# Autodesk Inventor assembly: Complete_leg_assembly
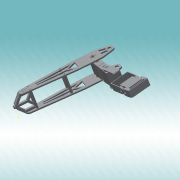
[picture p0: Inventor's stored thumbnail of the model, 180x180]
Saved by Autodesk Inventor 2019 (Build 230136000, 136)
## iProperties
Created: 2019-02-07
Part Number: Complete_leg_assembly
Document SubType Name: Assembly
Designer: USUARIO
Author: USUARIO
## Documents named in this file (7)
- D:\Users\Documents\Inventor parts\Structure_Charlotte\Structure_Charlotte\Complete_leg_assembly.iam
- D:\Users\Documents\Inventor parts\Structure_Charlotte\Structure_Charlotte\Motor_assembly.iam
- D:\Users\Documents\Inventor parts\Structure_Charlotte\Structure_Charlotte\SHEET_METAL1.ipt
- D:\Users\Documents\Inventor parts\Structure_Charlotte\Structure_Charlotte\SHEET_METAL2.ipt
- D:\Users\Documents\Inventor parts\Structure_Charlotte\Structure_Charlotte\Motor.ipt
- D:\Users\Documents\Inventor parts\Structure_Charlotte\Structure_Charlotte\Motor_joint.ipt
- D:\Users\Documents\Inventor parts\Structure_Charlotte\Structure_Charlotte\Leg_part3_variations\SHEET_METAL1_joint.ipt
## Components (14 placed, 7 different names)
1. Assembly_Leg:1 [sub-assembly] — Rotational:1
2. Motor_assembly:1 [sub-assembly] — Rotational:1, Rigid:1
3. SHEET_METAL1:1 — Rotational:2, Rigid:6
4. SHEET_METAL2:1 — Rigid:1, Rigid:2
5. SHEET_METAL2:2 — Rigid:2, Rigid:3
6. Motor:1 — Rigid:3, Rigid:4, Rigid:5
7. Motor_joint:1 — Rigid:5
8. Motor_joint:2 — Rigid:4, Rotational:2
9. SHEET_METAL1:2 — Rigid:6, Rotational:3
10. Motor:2 — Rigid:7, Rigid:8, Rigid:9
11. Motor_joint:3 — Rigid:8, Rotational:3
12. Motor_joint:4 — Rigid:7
13. SHEET_METAL2:3 — Rigid:9, Rigid:10
14. SHEET_METAL1_joint:1 — Rigid:10
## Relationships (13: WeldJoint 10, RevoluteJoint 3)
- Rotational:1 [RevoluteJoint]: Assembly_Leg:1 ↔ Motor_assembly:1
- Rigid:1 [WeldJoint]: Motor_assembly:1 ↔ SHEET_METAL2:1
- Rigid:2 [WeldJoint]: SHEET_METAL2:1 ↔ SHEET_METAL2:2
- Rigid:3 [WeldJoint]: SHEET_METAL2:2 ↔ Motor:1
- Rigid:4 [WeldJoint]: Motor:1 ↔ Motor_joint:2
- Rigid:5 [WeldJoint]: Motor:1 ↔ Motor_joint:1
- Rotational:2 [RevoluteJoint]: SHEET_METAL1:1 ↔ Motor_joint:2
- Rigid:6 [WeldJoint]: SHEET_METAL1:1 ↔ SHEET_METAL1:2
- Rigid:7 [WeldJoint]: Motor:2 ↔ Motor_joint:4
- Rigid:8 [WeldJoint]: Motor:2 ↔ Motor_joint:3
- Rotational:3 [RevoluteJoint]: SHEET_METAL1:2 ↔ Motor_joint:3
- Rigid:9 [WeldJoint]: Motor:2 ↔ SHEET_METAL2:3
- Rigid:10 [WeldJoint]: SHEET_METAL2:3 ↔ SHEET_METAL1_joint:1
